# Autodesk Inventor assembly: Assemblyfull
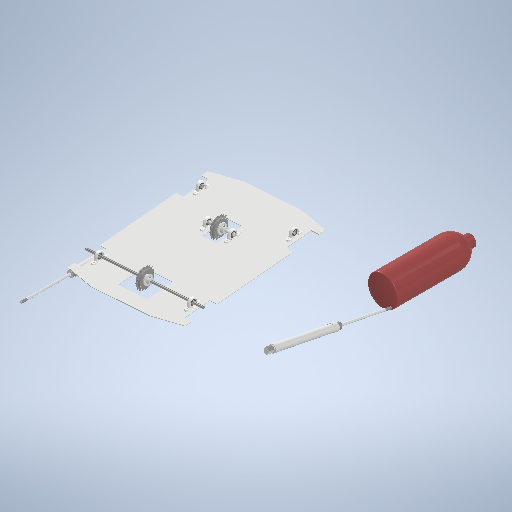
[picture p0: Inventor's stored thumbnail of the model, 512x512]
Saved by Autodesk Inventor 2026.1 (Build 301233020, 233B)
## iProperties
Created: 2026-01-22
Part Number: Assemblyfull
Document SubType Name: Assembly
Designer: user
Author: user
## Documents named in this file (7)
- D:\asu\machine element design\project\design\Assemblyfull.iam
- D:\asu\machine element design\project\design\chassis.ipt
- C:\Users\user\Downloads\pillow-block-bearing-p08-1.snapshot.17\Pillow Block P08\Pillow Block P08\Pillow Block P08.ipt
- D:\asu\machine element design\project\design\shaft assembly.iam
- D:\asu\machine element design\project\design\Assemblyfree gear.iam
- D:\asu\machine element design\project\design\piston\piston .iam
- D:\asu\machine element design\project\design\tank.ipt
## Components (12 placed, 6 different names)
1. chassis:1 — Mate:1, Mate:2, Mate:3, Mate:4, Mate:5, Mate:6, Mate:7, Mate:8, Mate:9, Mate:10, Mate:11, Mate:12, Mate:14, Mate:15, Mate:16, Mate:17, Mate:18, Mate:19
2. Pillow Block P08:1 — Mate:1, Mate:2, Mate:3
3. Pillow Block P08:2 — Mate:5, Mate:11, Mate:12
4. Pillow Block P08:3 — Mate:6, Mate:7, Mate:8, Mate:13
5. Pillow Block P08:4 — Mate:4, Mate:9, Mate:10
6. shaft assembly:1 [sub-assembly] — Mate:13
7. Pillow Block P08:5 — Mate:15, Mate:16, Mate:17
8. Pillow Block P08:6 — Mate:14, Mate:18, Mate:19, Mate:20
9. Assemblyfree gear:1 [sub-assembly] — Mate:20
10. piston :1 [sub-assembly]
11. piston :2 [sub-assembly]
12. tank:1
## Relationships (20: Mate 20)
- Mate:1: chassis:1 ↔ Pillow Block P08:1
- Mate:2: chassis:1 ↔ Pillow Block P08:1
- Mate:3: chassis:1 ↔ Pillow Block P08:1
- Mate:4: chassis:1 ↔ Pillow Block P08:4
- Mate:5: chassis:1 ↔ Pillow Block P08:2
- Mate:6: chassis:1 ↔ Pillow Block P08:3
- Mate:7: chassis:1 ↔ Pillow Block P08:3
- Mate:8: chassis:1 ↔ Pillow Block P08:3
- Mate:9: chassis:1 ↔ Pillow Block P08:4
- Mate:10: chassis:1 ↔ Pillow Block P08:4
- Mate:11: chassis:1 ↔ Pillow Block P08:2
- Mate:12: chassis:1 ↔ Pillow Block P08:2
- Mate:13: Pillow Block P08:3 ↔ shaft assembly:1
- Mate:14: chassis:1 ↔ Pillow Block P08:6
- Mate:15: chassis:1 ↔ Pillow Block P08:5
- Mate:16: chassis:1 ↔ Pillow Block P08:5
- Mate:17: chassis:1 ↔ Pillow Block P08:5
- Mate:18: chassis:1 ↔ Pillow Block P08:6
- Mate:19: chassis:1 ↔ Pillow Block P08:6
- Mate:20: Pillow Block P08:6 ↔ Assemblyfree gear:1
